# Autodesk Inventor assembly: DribblerUnit
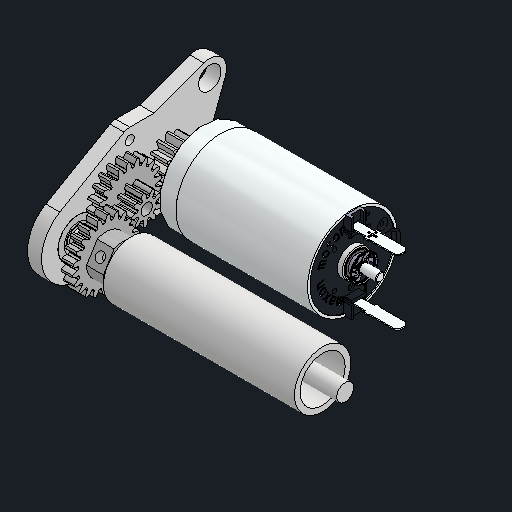
[picture p0: Inventor's stored thumbnail of the model, 512x512]
Saved by Autodesk Inventor 2024.2 (Build 282272000, 272)
## iProperties
Created: 2023-12-27
Part Number: DribblerUnit
Document SubType Name: Assembly
Designer: Hanaoka
Author: Hanaoka
## Documents named in this file (9)
- G:\共有ドライブ\reRo\05_個人\hanaoka\inventor\DribblerUnit\DribblerUnit.iam
- G:\共有ドライブ\reRo\05_個人\hanaoka\inventor\HandleUnit\GearCover.ipt
- G:\共有ドライブ\reRo\05_個人\hanaoka\inventor\DribblerUnit\Shaft.ipt
- G:\共有ドライブ\reRo\05_個人\hanaoka\inventor\DribblerUnit\Bearing_C-FL673ZZ.ipt
- G:\共有ドライブ\reRo\05_個人\hanaoka\inventor\DribblerUnit\dcx16s\dcx16s.iam
- G:\共有ドライブ\reRo\05_個人\hanaoka\inventor\DribblerUnit\DS0_5-12_On.ipt
- G:\共有ドライブ\reRo\05_個人\hanaoka\inventor\DribblerUnit\Gear_M0.5_22th.ipt
- G:\共有ドライブ\reRo\05_個人\hanaoka\inventor\DribblerUnit\Gear_M0.5_9th_21th.ipt
- G:\共有ドライブ\reRo\05_個人\hanaoka\inventor\DribblerUnit\tube.ipt
## Components (8 placed, 8 different names)
1. GearCover:1 — 挿入:1, 挿入:4, 挿入:5
2. Shaft:1 — 挿入:2
3. Bearing_C-FL673ZZ:1 — 挿入:1, 挿入:2
4. dcx16s:1 [sub-assembly] — 挿入:3
5. DS0_5-12_On:1 — 挿入:3
6. Gear_M0.5_22th:1 — 挿入:5, 挿入:6
7. Gear_M0.5_9th_21th:1 — 挿入:4
8. tube:1 — 挿入:6
## Relationships (6: Insert 6)
- 挿入:1 [Insert]: GearCover:1 ↔ Bearing_C-FL673ZZ:1
- 挿入:2 [Insert]: Shaft:1 ↔ Bearing_C-FL673ZZ:1
- 挿入:3 [Insert]: dcx16s:1 ↔ DS0_5-12_On:1
- 挿入:4 [Insert] (0.5 mm): GearCover:1 ↔ Gear_M0.5_9th_21th:1
- 挿入:5 [Insert] (3 mm): GearCover:1 ↔ Gear_M0.5_22th:1
- 挿入:6 [Insert] (1.5 mm): Gear_M0.5_22th:1 ↔ tube:1
